# Autodesk Inventor assembly: Assembly1
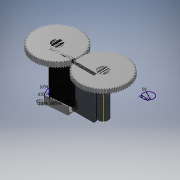
[picture p0: Inventor's stored thumbnail of the model, 180x180]
Saved by Autodesk Inventor 2019 (Build 230136000, 136)
## iProperties
Created: 2020-04-03
Part Number: Assembly1
Document SubType Name: Assembly
Designer: laca
_SolveAssemblyDoc: Frame Generator Solve Assembly
_Version: 15.0.0
Author: laca
## Documents named in this file (5)
- C:\Users\laca\Documents\Inventor\KeziVakolo\Assembly1.iam
- C:\Users\laca\Documents\Inventor\KeziVakolo\kes.ipt
- C:\Users\laca\Documents\Inventor\KeziVakolo\Assembly1\Design Accelerator\Spur Gears1.iam
- C:\Users\laca\Documents\Inventor\KeziVakolo\Part7.ipt
- C:\Users\laca\Documents\Inventor\KeziVakolo\Assembly1\Frame\Frame0001.iam
## Components (5 placed, 4 different names)
1. kes:1 — Rigid:2, Mate:2, Flush:1
2. kes:2 — Rigid:1, Mate:1, Flush:1
3. Spur Gears:1 [sub-assembly] — Rigid:1, Rigid:2
4. Part7:1
5. Frame0001:1 [sub-assembly]
## Relationships (5: WeldJoint 2, Mate 2, Flush 1)
- Rigid:1 [WeldJoint]: kes:2 ↔ Spur Gears:1
- Rigid:2 [WeldJoint]: kes:1 ↔ Spur Gears:1
- Mate:1: kes:2
- Mate:2: kes:1
- Flush:1: kes:1 ↔ kes:2
